# Autodesk Inventor assembly: Assem1
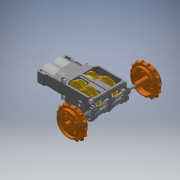
[picture p0: Inventor's stored thumbnail of the model, 180x180]
Saved by Autodesk Inventor 2019.1 (Build 231200000, 200)
## iProperties
Created: 2011-11-03
Part Number: Assem1
Document SubType Name: Assembly
Designer: poryz
Sending System: SolidWorks 2010
Last Author: Shebu
Last Saved: 2011-11-13
Author: poryz
## Documents named in this file (16)
- E:\Dropbox\_PRACA\HARDWARE\IE-TRACK-KIT-PWR-1\MECH\gearbox\Assem1.iam
- E:\Dropbox\_PRACA\HARDWARE\IE-TRACK-KIT-PWR-1\MECH\gearbox\middle.ipt
- E:\Dropbox\_PRACA\HARDWARE\IE-TRACK-KIT-PWR-1\MECH\gearbox\motor.ipt
- E:\Dropbox\_PRACA\HARDWARE\IE-TRACK-KIT-PWR-1\MECH\gearbox\left.ipt
- E:\Dropbox\_PRACA\HARDWARE\IE-TRACK-KIT-PWR-1\MECH\gearbox\right.ipt
- E:\Dropbox\_PRACA\HARDWARE\IE-TRACK-KIT-PWR-1\MECH\gearbox\DG_brass_gap4.0.ipt
- E:\Dropbox\_PRACA\HARDWARE\IE-TRACK-KIT-PWR-1\MECH\gearbox\DG_gold_brass.ipt
- E:\Dropbox\_PRACA\HARDWARE\IE-TRACK-KIT-PWR-1\MECH\gearbox\DG_purple_8_mtr.ipt
- E:\Dropbox\_PRACA\HARDWARE\IE-TRACK-KIT-PWR-1\MECH\gearbox\DG_shaft_23mm.ipt
- E:\Dropbox\_PRACA\HARDWARE\IE-TRACK-KIT-PWR-1\MECH\gearbox\DG_shaft_50mm.ipt
- E:\Dropbox\_PRACA\HARDWARE\IE-TRACK-KIT-PWR-1\MECH\gearbox\DG_yellow_34_12_N01.ipt
- E:\Dropbox\_PRACA\HARDWARE\IE-TRACK-KIT-PWR-1\MECH\gearbox\TG_G3.ipt
- E:\Dropbox\_PRACA\HARDWARE\IE-TRACK-KIT-PWR-1\MECH\gearbox\TG_G2.ipt
- E:\Dropbox\_PRACA\HARDWARE\IE-TRACK-KIT-PWR-1\MECH\gearbox\middle pin.ipt
- E:\Dropbox\_PRACA\HARDWARE\IE-TRACK-KIT-PWR-1\MECH\gearbox\Pan Head Cross Recess Screw_DIN.ipt
- E:\Dropbox\_PRACA\HARDWARE\IE-TRACK-KIT-PWR-1\MECH\wheels\drive sprocket.ipt
## Components (43 placed, 15 different names)
1. middle:1 — Mate:1, Mate:2
2. motor:1
3. left:1
4. right:1
5. motor:2
6. DG_brass_gap4.0:1
7. DG_gold_brass:1
8. DG_purple_8_mtr:1
9. DG_shaft_23mm:1
10. DG_shaft_50mm:1 — Mate:1, Rigid:1
11. DG_yellow_34_12_N01:1
12. TG_G3:2
13. DG_purple_8_mtr:2
14. DG_brass_gap4.0:2
15. DG_brass_gap4.0:3
16. DG_shaft_23mm:2
17. DG_brass_gap4.0:5
18. DG_brass_gap4.0:6
19. DG_brass_gap4.0:7
20. DG_brass_gap4.0:8
21. DG_brass_gap4.0:9
22. DG_brass_gap4.0:10
23. TG_G2:1
24. TG_G2:2
25. TG_G3:1
26. DG_shaft_50mm:2 — Mate:2, Rotational:1
27. DG_yellow_34_12_N01:2
28. TG_G2:3
29. TG_G2:4
30. DG_gold_brass:2
31. DG_brass_gap4.0:11
32. DG_brass_gap4.0:12
33. DG_brass_gap4.0:13
34. middle pin:3
35. middle pin:4
36. Pan head screw ISO 7045:1
37. Pan head screw ISO 7045:2
38. Pan head screw ISO 7045:3
39. Pan head screw ISO 7045:4
40. Pan head screw ISO 7045:5
41. Pan head screw ISO 7045:6
42. drive sprocket:1 — Rotational:1
43. drive sprocket:2 — Rigid:1
## Relationships (4: Mate 2, WeldJoint 1, RevoluteJoint 1)
- Mate:1 (-6 mm): middle:1 ↔ DG_shaft_50mm:1
- Mate:2 (-4 mm): middle:1 ↔ DG_shaft_50mm:2
- Rigid:1 [WeldJoint]: DG_shaft_50mm:1 ↔ drive sprocket:2
- Rotational:1 [RevoluteJoint]: DG_shaft_50mm:2 ↔ drive sprocket:1
